# Autodesk Inventor assembly: Rudder_Base
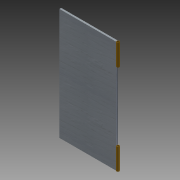
[picture p0: Inventor's stored thumbnail of the model, 180x180]
Saved by Autodesk Inventor 2011 SP1 (Build 150282100, 282)
## iProperties
Created: 2011-06-11
Part Number: Rudder_Base
Document SubType Name: Assembly
Designer: Andrew G. Meyer
Mass: 46.6823 g
Surface Area: 331.798 cm^2
Volume: 46.6823 cm^3
Density: 1 g/cm^3
Author: Andrew G. Meyer
## Documents named in this file (3)
- C:\Users\Andrew G. Meyer\Documents\Inventor\Hovercraft\Rudder_Base.iam
- C:\Users\Andrew G. Meyer\Documents\Inventor\Hovercraft\Rudder_Blade.ipt
- C:\Users\Andrew G. Meyer\Documents\Inventor\Hovercraft\Rudder_Hinge_Pipe.ipt
## Components (3 placed, 2 different names)
1. Rudder_Blade:1 — Insert:1, Insert:2
2. Rudder_Hinge_Pipe:1 — Insert:1
3. Rudder_Hinge_Pipe:2 — Insert:2
## Relationships (2: Insert 2)
- Insert:1: Rudder_Blade:1 ↔ Rudder_Hinge_Pipe:1
- Insert:2: Rudder_Blade:1 ↔ Rudder_Hinge_Pipe:2
